# Autodesk Inventor assembly: Assembly1
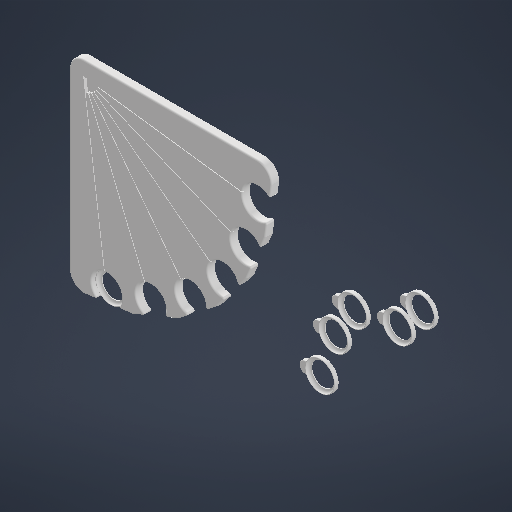
[picture p0: Inventor's stored thumbnail of the model, 512x512]
Saved by Autodesk Inventor 2026.2 (Build 302298000, 298)
## iProperties
Created: 2025-12-11
Part Number: Assembly1
Document SubType Name: Assembly
Designer: bubim
Author: bubim
## Documents named in this file (3)
- D:\CAD\Assembly1.iam
- D:\CAD\ShotFillerPlate.ipt
- D:\CAD\Shottfiller Adapter.ipt
## Components (7 placed, 2 different names)
1. ShotFillerPlate:1 — Mate:1, Mate:2
2. Shottfiller Adapter:2 — Mate:1, Mate:2
3. Shottfiller Adapter:3
4. Shottfiller Adapter:4
5. Shottfiller Adapter:5
6. Shottfiller Adapter:6
7. Shottfiller Adapter:7
## Relationships (2: Mate 2)
- Mate:1: ShotFillerPlate:1 ↔ Shottfiller Adapter:2
- Mate:2: ShotFillerPlate:1 ↔ Shottfiller Adapter:2
